# Autodesk Inventor assembly: Laptop
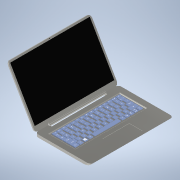
[picture p0: Inventor's stored thumbnail of the model, 180x180]
Saved by Autodesk Inventor 2022 (Build 260153000, 153)
## iProperties
Created: 2023-01-03
Part Number: Laptop
Document SubType Name: Assembly
Designer: mihir
Author: mihir
## Documents named in this file (3)
- C:\Users\mihir\Documents\Personal\InventorBuilds\Laptop.iam
- C:\Users\mihir\Documents\Personal\InventorBuilds\Room\LaptopBase.ipt
- C:\Users\mihir\Documents\Personal\InventorBuilds\Room\LaptopScreen.ipt
## Components (2 placed, 2 different names)
1. LaptopBase:1 — Angle:1, Flush:1, Mate:1
2. LaptopScreen:1 — Angle:1, Flush:1, Mate:1
## Relationships (3: Angle 1, Flush 1, Mate 1)
- Angle:1 (300 deg): LaptopBase:1 ↔ LaptopScreen:1
- Flush:1: LaptopBase:1 ↔ LaptopScreen:1
- Mate:1: LaptopBase:1 ↔ LaptopScreen:1
